# Autodesk Inventor assembly: High Strength 60-tooth Gear-Free Spinning Insert
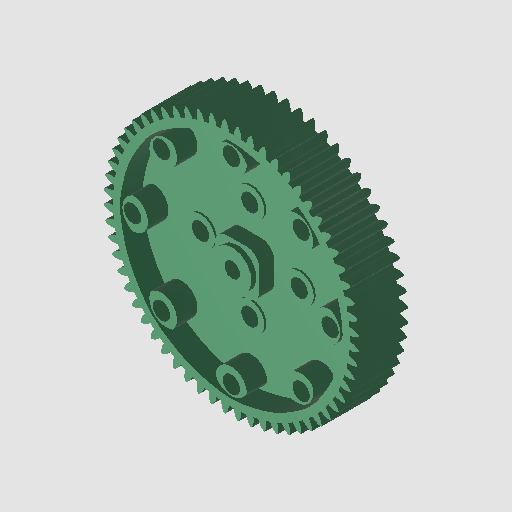
[picture p0: Inventor's stored thumbnail of the model, 512x512]
Saved by Autodesk Inventor 2019.4 (Build 234330000, 330)
## iProperties
Category: Motion
Company: Super Sonic Sparks, Team 24
Document SubType Name: Assembly
Designer: Jordan Kiesel
Description: High strength free spinning idler gear.
Vendor: VEX Robotics, Inc.
Catalog Web Link: http://www.vexrobotics.com/products/accessories/motion/276-2250.html
Mass: 22.6681 g
Surface Area: 174.277 cm^2
Volume: 15.9075 cm^3
Density: 1.425 g/cm^3
Created: 2019-07-01
Author: Jordan Kiesel
Title: High Strength 60-tooth Gear-Free Spinning Insert
Comments: Build mechanisms capable of withstanding higher stresses than ever before. Lift heavier loads, and survive bigger impacts with high strength gears. ▷ High strength gears mate with all VEX spur gears. ▷ Double-thick face width provides added tooth strength. ▷ Use the round-hole inserts to build free spinning idler gears. ▷ Build gearboxes that resist high shock-loads. ▷ Bolt Gears together for added strength.
## Documents named in this file (3)
- C:\Users\Citru\Documents\SID Library-20190630T175114Z-001\2018 BNS-VRC-SID Library\Motion\Spur Gears\High Strength 60-tooth Gear, Free Spinning Insert.iam
- C:\Users\Citru\Documents\SID Library-20190630T175114Z-001\2018 BNS-VRC-SID Library\Motion\Spur Gears\Reference Parts\High Strength Gears\High Strength 60-Tooth Gear.ipt
- C:\Users\Citru\Documents\SID Library-20190630T175114Z-001\2018 BNS-VRC-SID Library\Motion\Reference Parts\Free Spinning Gear Insert.ipt
## Components (3 placed, 2 different names)
1. High Strength 60-Tooth Gear:1 — Mate:1, Mate:2, Mate:3, Mate:4, Mate:5, Mate:6
2. Free Spinning Gear Insert:1 — Mate:1, Mate:2, Mate:3
3. Free Spinning Gear Insert:2 — Mate:4, Mate:5, Mate:6
## Relationships (6: Mate 6)
- Mate:1: High Strength 60-Tooth Gear:1 ↔ Free Spinning Gear Insert:1
- Mate:2 (0.0254 mm): High Strength 60-Tooth Gear:1 ↔ Free Spinning Gear Insert:1
- Mate:3 (0.0254 mm): High Strength 60-Tooth Gear:1 ↔ Free Spinning Gear Insert:1
- Mate:4: High Strength 60-Tooth Gear:1 ↔ Free Spinning Gear Insert:2
- Mate:5 (0.0254 mm): High Strength 60-Tooth Gear:1 ↔ Free Spinning Gear Insert:2
- Mate:6 (0.0254 mm): High Strength 60-Tooth Gear:1 ↔ Free Spinning Gear Insert:2
